# Autodesk Inventor assembly: jigAndRunnerAssembly
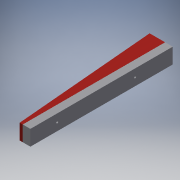
[picture p0: Inventor's stored thumbnail of the model, 180x180]
Saved by Autodesk Inventor 2019.1 (Build 231200000, 200)
## iProperties
Created: 2018-08-02
Part Number: jigAndRunnerAssembly
Document SubType Name: Assembly
Designer: steele
Author: steele
## Documents named in this file (3)
- C:\git\CAD-Development\robSteele\HouseProjects\TableSaw\jigAndRunnerAssembly.iam
- C:\git\CAD-Development\robSteele\HouseProjects\TableSaw\tableSawRunner.ipt
- C:\git\CAD-Development\robSteele\HouseProjects\TableSaw\jigForRipCuts.ipt
## Components (2 placed, 2 different names)
1. tableSawRunner:1 — Insert:1, Insert:2
2. jigForRipCuts:1 — Insert:1, Insert:2
## Relationships (2: Insert 2)
- Insert:1: tableSawRunner:1 ↔ jigForRipCuts:1
- Insert:2: tableSawRunner:1 ↔ jigForRipCuts:1
